# Autodesk Inventor assembly: shooting Mechanism
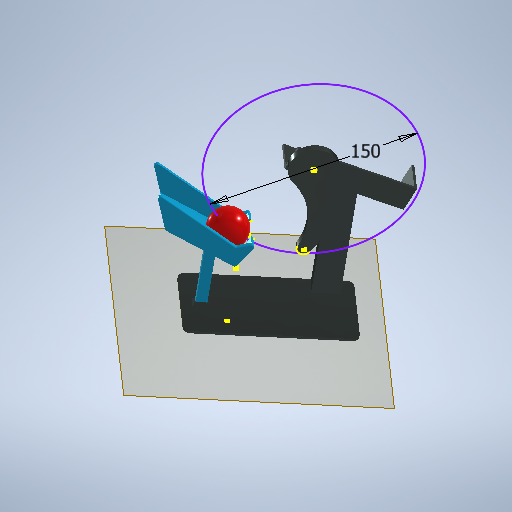
[picture p0: Inventor's stored thumbnail of the model, 512x512]
Saved by Autodesk Inventor 2025.4 (Build 294407000, 407)
## iProperties
Created: 2026-03-03
Part Number: shooting Mechanism
Document SubType Name: Assembly
Designer: youse
Author: youse
## Documents named in this file (5)
- D:\basics project\shooting Mechanism.iam
- D:\basics project\shaft.ipt
- D:\basics project\shooter.ipt
- D:\basics project\shooting slider.ipt
- D:\basics project\testing ball.ipt
## Components (4 placed, 4 different names)
1. shaft:1 — Mate:1, Mate:2
2. shooter:1 — Mate:2, Mate:3
3. shooting slider:1 — Mate:1, Mate:3
4. testing ball:1
## Relationships (3: Mate 3)
- Mate:1: shaft:1 ↔ shooting slider:1
- Mate:2: shaft:1 ↔ shooter:1
- Mate:3: shooter:1 ↔ shooting slider:1
